# Autodesk Inventor assembly: KN-00-01-00
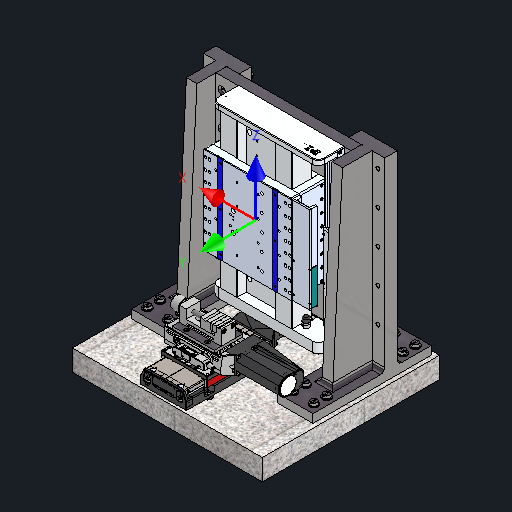
[picture p0: Inventor's stored thumbnail of the model, 512x512]
Saved by Autodesk Inventor 2025.2 (Build 292293000, 293)
## iProperties
Created: 2025-01-15
Part Number: KN-00-01-00
Document SubType Name: Assembly
Designer: Kacper Mik
Author: Kacper Mik
## Documents named in this file (20)
- C:\Users\kacpe\Documents\STUDIA\INŻYNIERKA\Nanotwardościomierz\Nanotwardosciomierz inventor\00-01-zesp_podstawy.iam
- 01-00-zesp_podstawy.iam
- C:\Users\kacpe\Documents\STUDIA\INŻYNIERKA\Nanotwardościomierz\Nanotwardosciomierz inventor\00-01-Podstawa.ipt
- C:\Users\kacpe\Documents\STUDIA\INŻYNIERKA\Nanotwardościomierz\Nanotwardosciomierz inventor\Pobrane\L-509.033111\L-509.033111\L-509.033111.ipt
- C:\Users\kacpe\Documents\STUDIA\INŻYNIERKA\Nanotwardościomierz\Nanotwardosciomierz inventor\Pobrane\L-511.033111\L-511.033111.ipt
- C:\Users\kacpe\Documents\STUDIA\INŻYNIERKA\Nanotwardościomierz\Nanotwardosciomierz inventor\CC\en-US\ISO 1207(2)\ISO 1207 - M4 x 14.ipt
- C:\Users\kacpe\Documents\STUDIA\INŻYNIERKA\Nanotwardościomierz\Nanotwardosciomierz inventor\Nogi\wkladka do nog.ipt
- C:\Users\kacpe\Documents\STUDIA\INŻYNIERKA\Nanotwardościomierz\Nanotwardosciomierz inventor\Nogi\noga.ipt
- C:\Users\kacpe\Documents\STUDIA\INŻYNIERKA\Nanotwardościomierz\Nanotwardosciomierz inventor\Part1.ipt
- C:\Users\kacpe\Documents\STUDIA\INŻYNIERKA\Nanotwardościomierz\Nanotwardosciomierz inventor\Pobrane\imadlo\AIS2024\33225-10-353210.iam
- C:\Users\kacpe\Documents\STUDIA\INŻYNIERKA\Nanotwardościomierz\Nanotwardosciomierz inventor\CC\en-US\ISO 1207(2)\ISO 1207 - M6 x 10.ipt
- C:\Users\kacpe\Documents\STUDIA\INŻYNIERKA\Nanotwardościomierz\Nanotwardosciomierz inventor\CC\en-US\ISO 1207(2)\ISO 1207 - M6 x 12.ipt
- C:\Users\kacpe\Documents\STUDIA\INŻYNIERKA\Nanotwardościomierz\Nanotwardosciomierz inventor\Pobrane\A-123.100x1_PIGLIDE AT3 AIR BEARING STAGE, 100MM\A-123.100x1_PIGLIDE AT3 AIR BEARING STAGE, 100MM.ipt
- C:\Users\kacpe\Documents\STUDIA\INŻYNIERKA\Nanotwardościomierz\Nanotwardosciomierz inventor\01-03-Plyta_stolika_Z.ipt
- C:\Users\kacpe\Documents\STUDIA\INŻYNIERKA\Nanotwardościomierz\Nanotwardosciomierz inventor\01-04-podpora.ipt
- C:\Users\kacpe\Documents\STUDIA\INŻYNIERKA\Nanotwardościomierz\Nanotwardosciomierz inventor\01-04-podpora_MIR.ipt
- C:\Users\kacpe\Documents\STUDIA\INŻYNIERKA\Nanotwardościomierz\Nanotwardosciomierz inventor\CC\en-US\ISO 1207(2)\ISO 1207 - M10 x 60.ipt
- C:\Users\kacpe\Documents\STUDIA\INŻYNIERKA\Nanotwardościomierz\Nanotwardosciomierz inventor\CC\en-US\ISO 4161\ISO 4161 - M10(1).ipt
- C:\Users\kacpe\Documents\STUDIA\INŻYNIERKA\Nanotwardościomierz\Nanotwardosciomierz inventor\CC\en-US\ISO 7089\ISO 7089 - 10 - 140 HV(1).ipt
- C:\Users\kacpe\Documents\STUDIA\INŻYNIERKA\Nanotwardościomierz\Nanotwardosciomierz inventor\CC\en-US\ISO 1207(2)\ISO 1207 - M5 x 10.ipt
## Components (87 placed, 19 different names)
1. 01-01-Podstawa:1 — Angle:6, Insert:10, Mate:6, Angle:8, Insert:26, Insert:27, Insert:28, Insert:29, WAZNE WYSOKOSC Z, Mate:11
2. 01-02-podkladka_imadlo — Insert:16, Insert:17, Insert:18, Insert:19, Insert:20, Insert:21, Insert:22, Insert:23, Insert:24, Insert:25
3. 01-03-Plyta_stolika_Z:1 — Insert:36, Insert:37, WAZNE WYSOKOSC Z, Mate:9, Mate:10, Mate:12, Mate:13, Mate:14, Mate:15, Mate:16, Mate:17, Mate:18, Mate:19, Mate:20, Mate:21, Mate:22, Mate:23, Mate:24, Mate:25, Mate:26, Mate:27, Mate:28, Mate:29, Mate:30, Mate:31, Mate:32, Mate:34, Mate:36, Mate:38, Mate:40, Mate:42, Mate:44, Mate:46, Mate:48, Mate:50
4. 01-04-podpora:1 — Mate:9, Mate:10, Mate:11, Mate:33, Mate:35, Mate:37, Mate:39, Mate:41, Mate:43, Mate:45, Mate:47, Mate:49, Mate:51, Mate:52, Mate:53, Mate:54, Mate:55, Mate:56, Mate:57, Mate:58, Mate:59, Mate:60, Mate:61, Mate:62, Mate:63, Mate:64, Mate:65, Mate:66, Mate:67
5. 01-04-podpora_MIR:1
6. ISO 1207 M10 x 60:1 — Mate:12, Mate:13
7. ISO 4161 M10:1 — Mate:32, Mate:33
8. ISO 1207 M10 x 60:2 — Mate:14, Mate:15
9. ISO 1207 M10 x 60:3 — Mate:16, Mate:17
10. ISO 1207 M10 x 60:4 — Mate:18, Mate:19
11. ISO 1207 M10 x 60:5 — Mate:20, Mate:21
12. ISO 1207 M10 x 60:6 — Mate:22, Mate:23
13. ISO 1207 M10 x 60:7 — Mate:24, Mate:25
14. ISO 1207 M10 x 60:8 — Mate:26, Mate:27
15. ISO 1207 M10 x 60:9 — Mate:28, Mate:29
16. ISO 1207 M10 x 60:10 — Mate:30, Mate:31
17. ISO 4161 M10:2 — Mate:34, Mate:35
18. ISO 4161 M10:3 — Mate:36, Mate:37
19. ISO 4161 M10:4 — Mate:38, Mate:39
20. ISO 4161 M10:5 — Mate:40, Mate:41
21. ISO 4161 M10:6 — Mate:42, Mate:43
22. ISO 4161 M10:7 — Mate:44, Mate:45
23. ISO 4161 M10:8 — Mate:46, Mate:47
24. ISO 4161 M10:9 — Mate:48, Mate:49
25. ISO 4161 M10:10 — Mate:50, Mate:51
26. ISO 7089 10:1 — Mate:52, Mate:53, Insert:38
27. ISO 1207 M10 x 60:11 — Insert:38
28. ISO 7089 10:2 — Mate:54, Mate:55, Insert:39
29. ISO 7089 10:3 — Mate:56, Mate:57, Insert:40
30. ISO 7089 10:4 — Mate:58, Mate:59, Insert:41
31. ISO 7089 10:5 — Mate:60, Mate:61, Insert:42
32. ISO 7089 10:6 — Mate:62, Mate:63, Insert:43
33. ISO 7089 10:7 — Mate:64, Mate:65, Insert:44
34. ISO 7089 10:8 — Mate:66, Mate:67, Insert:45
35. ISO 1207 M10 x 60:12 — Insert:39
36. ISO 1207 M10 x 60:13 — Insert:40
37. ISO 1207 M10 x 60:14 — Insert:41
38. ISO 1207 M10 x 60:15 — Insert:42
39. ISO 1207 M10 x 60:16 — Insert:43
40. ISO 1207 M10 x 60:17 — Insert:44
41. ISO 1207 M10 x 60:18 — Insert:45
42. ISO 7089 10:9 — Insert:46
43. ISO 1207 M10 x 60:19 — Insert:46
44. ISO 7089 10:10 — Insert:47
45. ISO 7089 10:11 — Insert:48
46. ISO 7089 10:12 — Insert:49
47. ISO 7089 10:13 — Insert:50
48. ISO 7089 10:14 — Insert:51
49. ISO 7089 10:15 — Insert:52
50. ISO 7089 10:16 — Insert:53
51. ISO 1207 M10 x 60:20 — Insert:47
52. ISO 1207 M10 x 60:21 — Insert:48
53. ISO 1207 M10 x 60:22 — Insert:49
54. ISO 1207 M10 x 60:23 — Insert:50
55. ISO 1207 M10 x 60:24 — Insert:51
56. ISO 1207 M10 x 60:25 — Insert:52
57. ISO 1207 M10 x 60:26 — Insert:53
58. A-123.100x1_PIGLIDE AT3 AIR BEARING STAGE, 100MM:1 — Angle:9, Mate:7, Insert:36, Insert:37, Flush:13
59. 33225-10-353210:1 [sub-assembly] — Insert:16, Insert:17
60. L-511.033111:1 — Angle:5, Angle:6, Angle:7, Insert:9, Insert:30, Insert:31, Insert:32, Insert:33, Insert:34, Insert:35
61. L-509.033111:1 — Angle:2, Angle:7, Insert:5, Insert:6, Insert:7, Insert:8, Insert:9, Insert:20, Insert:21
62. wkladka do nog:8 — Insert:27
63. wkladka do nog:7 — Insert:29
64. wkladka do nog:6 — Insert:28, Insert:31
65. wkladka do nog:5 — Insert:26, Insert:30
66. ISO 1207 M6 x 12:4 — Insert:34
67. ISO 1207 M6 x 12:3 — Insert:32
68. ISO 1207 M6 x 12:2 — Insert:35
69. ISO 1207 M6 x 12:1 — Insert:33
70. ISO 1207 M4 x 14:4 — Insert:5
71. ISO 1207 M4 x 14:3 — Insert:8
72. ISO 1207 M4 x 14:2 — Insert:7
73. ISO 1207 M4 x 14:1 — Insert:6
74. ISO 1207 M6 x 10:4 — Insert:25
75. ISO 1207 M6 x 10:3 — Insert:23
76. ISO 1207 M6 x 10:2 — Insert:22
77. ISO 1207 M6 x 10:1 — Insert:24
78. ISO 1207 M5 x 10:1 — Insert:19
79. ISO 1207 M5 x 10:2 — Insert:18
80. wkladka granit M6:1 — Insert:10, Insert:11
81. noga:1 — Insert:11
82. wkladka do nog:2
83. noga:2
84. wkladka do nog:3
85. noga:3
86. wkladka do nog:4
87. noga:4
## Component patterns: (4 elements, first: wkladka granit M6:1 + noga:1)
## Relationships (114: Mate 62, Insert 45, Angle 6, Flush 1)
- Angle:2 (180 deg): L-509.033111:1
- Angle:5 (0 deg): L-511.033111:1
- Angle:6 (0 deg): 01-01-Podstawa:1 ↔ L-511.033111:1
- Angle:7 (0 deg): L-511.033111:1 ↔ L-509.033111:1
- Insert:5: L-509.033111:1 ↔ ISO 1207 M4 x 14:4
- Insert:6: L-509.033111:1 ↔ ISO 1207 M4 x 14:1
- Insert:7: L-509.033111:1 ↔ ISO 1207 M4 x 14:2
- Insert:8: L-509.033111:1 ↔ ISO 1207 M4 x 14:3
- Insert:9: L-511.033111:1 ↔ L-509.033111:1
- Insert:10: 01-01-Podstawa:1 ↔ wkladka granit M6:1
- Insert:11: wkladka granit M6:1 ↔ noga:1
- Mate:6: 01-01-Podstawa:1
- Angle:8 (0 deg): 01-01-Podstawa:1
- Insert:16: 01-02-podkladka_imadlo ↔ 33225-10-353210:1
- Insert:17: 01-02-podkladka_imadlo ↔ 33225-10-353210:1
- Insert:18: 01-02-podkladka_imadlo ↔ ISO 1207 M5 x 10:2
- Insert:19: 01-02-podkladka_imadlo ↔ ISO 1207 M5 x 10:1
- Insert:20: 01-02-podkladka_imadlo ↔ L-509.033111:1
- Insert:21: 01-02-podkladka_imadlo ↔ L-509.033111:1
- Insert:22: 01-02-podkladka_imadlo ↔ ISO 1207 M6 x 10:2
- Insert:23: 01-02-podkladka_imadlo ↔ ISO 1207 M6 x 10:3
- Insert:24: 01-02-podkladka_imadlo ↔ ISO 1207 M6 x 10:1
- Insert:25: 01-02-podkladka_imadlo ↔ ISO 1207 M6 x 10:4
- Insert:26: 01-01-Podstawa:1 ↔ wkladka do nog:5
- Insert:27: 01-01-Podstawa:1 ↔ wkladka do nog:8
- Insert:28: 01-01-Podstawa:1 ↔ wkladka do nog:6
- Insert:29: 01-01-Podstawa:1 ↔ wkladka do nog:7
- Insert:30: L-511.033111:1 ↔ wkladka do nog:5
- Insert:31: L-511.033111:1 ↔ wkladka do nog:6
- Insert:32: L-511.033111:1 ↔ ISO 1207 M6 x 12:3
- Insert:33: L-511.033111:1 ↔ ISO 1207 M6 x 12:1
- Insert:34: L-511.033111:1 ↔ ISO 1207 M6 x 12:4
- Insert:35: L-511.033111:1 ↔ ISO 1207 M6 x 12:2
- Angle:9 (0 deg): A-123.100x1_PIGLIDE AT3 AIR BEARING STAGE, 100MM:1
- Mate:7: A-123.100x1_PIGLIDE AT3 AIR BEARING STAGE, 100MM:1
- Insert:36: 01-03-Plyta_stolika_Z:1 ↔ A-123.100x1_PIGLIDE AT3 AIR BEARING STAGE, 100MM:1
- Insert:37: 01-03-Plyta_stolika_Z:1 ↔ A-123.100x1_PIGLIDE AT3 AIR BEARING STAGE, 100MM:1
- WAZNE WYSOKOSC Z [Mate] (80 mm): 01-01-Podstawa:1 ↔ 01-03-Plyta_stolika_Z:1
- Mate:9: 01-03-Plyta_stolika_Z:1 ↔ 01-04-podpora:1
- Mate:10: 01-03-Plyta_stolika_Z:1 ↔ 01-04-podpora:1
- Mate:11: 01-01-Podstawa:1 ↔ 01-04-podpora:1
- Flush:13: A-123.100x1_PIGLIDE AT3 AIR BEARING STAGE, 100MM:1
- Mate:12: 01-03-Plyta_stolika_Z:1 ↔ ISO 1207 M10 x 60:1
- Mate:13: 01-03-Plyta_stolika_Z:1 ↔ ISO 1207 M10 x 60:1
- Mate:14: 01-03-Plyta_stolika_Z:1 ↔ ISO 1207 M10 x 60:2
- Mate:15: 01-03-Plyta_stolika_Z:1 ↔ ISO 1207 M10 x 60:2
- Mate:16: 01-03-Plyta_stolika_Z:1 ↔ ISO 1207 M10 x 60:3
- Mate:17: 01-03-Plyta_stolika_Z:1 ↔ ISO 1207 M10 x 60:3
- Mate:18: 01-03-Plyta_stolika_Z:1 ↔ ISO 1207 M10 x 60:4
- Mate:19: 01-03-Plyta_stolika_Z:1 ↔ ISO 1207 M10 x 60:4
- Mate:20: 01-03-Plyta_stolika_Z:1 ↔ ISO 1207 M10 x 60:5
- Mate:21: 01-03-Plyta_stolika_Z:1 ↔ ISO 1207 M10 x 60:5
- Mate:22: 01-03-Plyta_stolika_Z:1 ↔ ISO 1207 M10 x 60:6
- Mate:23: 01-03-Plyta_stolika_Z:1 ↔ ISO 1207 M10 x 60:6
- Mate:24: 01-03-Plyta_stolika_Z:1 ↔ ISO 1207 M10 x 60:7
- Mate:25: 01-03-Plyta_stolika_Z:1 ↔ ISO 1207 M10 x 60:7
- Mate:26: 01-03-Plyta_stolika_Z:1 ↔ ISO 1207 M10 x 60:8
- Mate:27: 01-03-Plyta_stolika_Z:1 ↔ ISO 1207 M10 x 60:8
- Mate:28: 01-03-Plyta_stolika_Z:1 ↔ ISO 1207 M10 x 60:9
- Mate:29: 01-03-Plyta_stolika_Z:1 ↔ ISO 1207 M10 x 60:9
- Mate:30: 01-03-Plyta_stolika_Z:1 ↔ ISO 1207 M10 x 60:10
- Mate:31: 01-03-Plyta_stolika_Z:1 ↔ ISO 1207 M10 x 60:10
- Mate:32: 01-03-Plyta_stolika_Z:1 ↔ ISO 4161 M10:1
- Mate:33: 01-04-podpora:1 ↔ ISO 4161 M10:1
- Mate:34: 01-03-Plyta_stolika_Z:1 ↔ ISO 4161 M10:2
- Mate:35: 01-04-podpora:1 ↔ ISO 4161 M10:2
- Mate:36: 01-03-Plyta_stolika_Z:1 ↔ ISO 4161 M10:3
- Mate:37: 01-04-podpora:1 ↔ ISO 4161 M10:3
- Mate:38: 01-03-Plyta_stolika_Z:1 ↔ ISO 4161 M10:4
- Mate:39: 01-04-podpora:1 ↔ ISO 4161 M10:4
- Mate:40: 01-03-Plyta_stolika_Z:1 ↔ ISO 4161 M10:5
- Mate:41: 01-04-podpora:1 ↔ ISO 4161 M10:5
- Mate:42: 01-03-Plyta_stolika_Z:1 ↔ ISO 4161 M10:6
- Mate:43: 01-04-podpora:1 ↔ ISO 4161 M10:6
- Mate:44: 01-03-Plyta_stolika_Z:1 ↔ ISO 4161 M10:7
- Mate:45: 01-04-podpora:1 ↔ ISO 4161 M10:7
- Mate:46: 01-03-Plyta_stolika_Z:1 ↔ ISO 4161 M10:8
- Mate:47: 01-04-podpora:1 ↔ ISO 4161 M10:8
- Mate:48: 01-03-Plyta_stolika_Z:1 ↔ ISO 4161 M10:9
- Mate:49: 01-04-podpora:1 ↔ ISO 4161 M10:9
- Mate:50: 01-03-Plyta_stolika_Z:1 ↔ ISO 4161 M10:10
- Mate:51: 01-04-podpora:1 ↔ ISO 4161 M10:10
- Mate:52: 01-04-podpora:1 ↔ ISO 7089 10:1
- Mate:53: 01-04-podpora:1 ↔ ISO 7089 10:1
- Mate:54: 01-04-podpora:1 ↔ ISO 7089 10:2
- Mate:55: 01-04-podpora:1 ↔ ISO 7089 10:2
- Mate:56: 01-04-podpora:1 ↔ ISO 7089 10:3
- Mate:57: 01-04-podpora:1 ↔ ISO 7089 10:3
- Mate:58: 01-04-podpora:1 ↔ ISO 7089 10:4
- Mate:59: 01-04-podpora:1 ↔ ISO 7089 10:4
- Mate:60: 01-04-podpora:1 ↔ ISO 7089 10:5
- Mate:61: 01-04-podpora:1 ↔ ISO 7089 10:5
- Mate:62: 01-04-podpora:1 ↔ ISO 7089 10:6
- Mate:63: 01-04-podpora:1 ↔ ISO 7089 10:6
- Mate:64: 01-04-podpora:1 ↔ ISO 7089 10:7
- Mate:65: 01-04-podpora:1 ↔ ISO 7089 10:7
- Mate:66: 01-04-podpora:1 ↔ ISO 7089 10:8
- Mate:67: 01-04-podpora:1 ↔ ISO 7089 10:8
- Insert:38: ISO 7089 10:1 ↔ ISO 1207 M10 x 60:11
- Insert:39: ISO 7089 10:2 ↔ ISO 1207 M10 x 60:12
- Insert:40: ISO 7089 10:3 ↔ ISO 1207 M10 x 60:13
- Insert:41: ISO 7089 10:4 ↔ ISO 1207 M10 x 60:14
- Insert:42: ISO 7089 10:5 ↔ ISO 1207 M10 x 60:15
- Insert:43: ISO 7089 10:6 ↔ ISO 1207 M10 x 60:16
- Insert:44: ISO 7089 10:7 ↔ ISO 1207 M10 x 60:17
- Insert:45: ISO 7089 10:8 ↔ ISO 1207 M10 x 60:18
- Insert:46: ISO 7089 10:9 ↔ ISO 1207 M10 x 60:19
- Insert:47: ISO 7089 10:10 ↔ ISO 1207 M10 x 60:20
- Insert:48: ISO 7089 10:11 ↔ ISO 1207 M10 x 60:21
- Insert:49: ISO 7089 10:12 ↔ ISO 1207 M10 x 60:22
- Insert:50: ISO 7089 10:13 ↔ ISO 1207 M10 x 60:23
- Insert:51: ISO 7089 10:14 ↔ ISO 1207 M10 x 60:24
- Insert:52: ISO 7089 10:15 ↔ ISO 1207 M10 x 60:25
- Insert:53: ISO 7089 10:16 ↔ ISO 1207 M10 x 60:26
